# Autodesk Inventor assembly: Omniwheel Assembly 1764
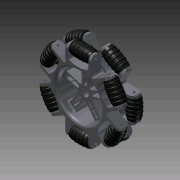
[picture p0: Inventor's stored thumbnail of the model, 180x180]
Saved by Autodesk Inventor 2011 (Build 150239000, 239)
## iProperties
Created: 2007-11-28
Part Number: Omniwheel Assembly 1764
Document SubType Name: Assembly
Designer: lwoods
Mass: 807.037 g
Surface Area: 1296.28 cm^2
Volume: 334.333 cm^3
Density: 2.41387 g/cm^3
Author: lwoods
## Documents named in this file (4)
- R:\CAD Archives\Wheels\Omniwheel\Omniwheel Assembly 1764.iam
- R:\CAD Archives\Wheels\Omniwheel\Omnidrive.ipt
- R:\CAD Archives\Wheels\Omniwheel\Roller Axle V4 1764.ipt
- R:\CAD Archives\Wheels\Omniwheel\roller assembly 1764.iam
## Components (25 placed, 3 different names)
1. Omnidrive:1 — Insert:1, Insert:2, Insert:3, Insert:4, Insert:5, Insert:6, Insert:7, Insert:8, Insert:9, Insert:10, Insert:11, Insert:12, Insert:16, Insert:17, Insert:19, Insert:20
2. Roller Axle V4 1764:1 — Insert:11, Insert:24
3. Roller Axle V4 1764:2 — Insert:8
4. Roller Axle V4 1764:3 — Insert:12, Insert:23
5. Roller Axle V4 1764:4 — Insert:10, Insert:22
6. Roller Axle V4 1764:5 — Insert:3, Insert:14
7. Roller Axle V4 1764:6 — Insert:4, Insert:18
8. Roller Axle V4 1764:7 — Insert:6
9. Roller Axle V4 1764:8 — Insert:2
10. Roller Axle V4 1764:9 — Insert:1, Insert:13
11. Roller Axle V4 1764:10 — Insert:5
12. Roller Axle V4 1764:11 — Insert:9, Insert:15
13. Roller Axle V4 1764:12 — Insert:7, Insert:21
14. roller assembly 1764:1 [sub-assembly] — Insert:18
15. roller assembly 1764:2 [sub-assembly] — Insert:20
16. roller assembly 1764:3 [sub-assembly] — Insert:17
17. roller assembly 1764:4 [sub-assembly] — Insert:19
18. roller assembly 1764:5 [sub-assembly] — Insert:21
19. roller assembly 1764:6 [sub-assembly] — Insert:22
20. roller assembly 1764:7 [sub-assembly] — Insert:23
21. roller assembly 1764:8 [sub-assembly] — Insert:24
22. roller assembly 1764:9 [sub-assembly] — Insert:16
23. roller assembly 1764:10 [sub-assembly] — Insert:15
24. roller assembly 1764:11 [sub-assembly] — Insert:13
25. roller assembly 1764:12 [sub-assembly] — Insert:14
## Relationships (24: Insert 24)
- Insert:1 (-45.8724 mm): Omnidrive:1 ↔ Roller Axle V4 1764:9
- Insert:2 (-45.8724 mm): Omnidrive:1 ↔ Roller Axle V4 1764:8
- Insert:3 (-45.8724 mm): Omnidrive:1 ↔ Roller Axle V4 1764:5
- Insert:4 (-45.8724 mm): Omnidrive:1 ↔ Roller Axle V4 1764:6
- Insert:5 (-45.8724 mm): Omnidrive:1 ↔ Roller Axle V4 1764:10
- Insert:6 (-45.8724 mm): Omnidrive:1 ↔ Roller Axle V4 1764:7
- Insert:7 (-45.8724 mm): Omnidrive:1 ↔ Roller Axle V4 1764:12
- Insert:8 (-45.8724 mm): Omnidrive:1 ↔ Roller Axle V4 1764:2
- Insert:9 (-45.8724 mm): Omnidrive:1 ↔ Roller Axle V4 1764:11
- Insert:10 (-45.8724 mm): Omnidrive:1 ↔ Roller Axle V4 1764:4
- Insert:11 (-45.8724 mm): Omnidrive:1 ↔ Roller Axle V4 1764:1
- Insert:12 (-45.8724 mm): Omnidrive:1 ↔ Roller Axle V4 1764:3
- Insert:13 (-40.132 mm): Roller Axle V4 1764:9 ↔ roller assembly 1764:11
- Insert:14 (-40.132 mm): Roller Axle V4 1764:5 ↔ roller assembly 1764:12
- Insert:15 (-40.132 mm): Roller Axle V4 1764:11 ↔ roller assembly 1764:10
- Insert:16 (-40.132 mm): Omnidrive:1 ↔ roller assembly 1764:9
- Insert:17 (-40.132 mm): Omnidrive:1 ↔ roller assembly 1764:3
- Insert:18 (-40.132 mm): Roller Axle V4 1764:6 ↔ roller assembly 1764:1
- Insert:19 (-40.132 mm): Omnidrive:1 ↔ roller assembly 1764:4
- Insert:20 (-40.132 mm): Omnidrive:1 ↔ roller assembly 1764:2
- Insert:21 (-40.132 mm): Roller Axle V4 1764:12 ↔ roller assembly 1764:5
- Insert:22 (-40.132 mm): Roller Axle V4 1764:4 ↔ roller assembly 1764:6
- Insert:23 (-40.132 mm): Roller Axle V4 1764:3 ↔ roller assembly 1764:7
- Insert:24 (-40.132 mm): Roller Axle V4 1764:1 ↔ roller assembly 1764:8
